# Autodesk Inventor assembly: Male straight header 15p
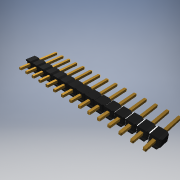
[picture p0: Inventor's stored thumbnail of the model, 180x180]
Saved by Autodesk Inventor 2017 (Build 210142000, 142)
## iProperties
Created: 2017-09-07
Part Number: Male straight header 15p
Document SubType Name: Assembly
Designer: denoqs
Author: denoqs
## Documents named in this file (3)
- E:\Graphic Development\Autodesk Inventor\Inventor output\Arduino things\Arduino header\Male straight header 15p.iam
- E:\Graphic Development\Autodesk Inventor\Inventor output\Arduino things\Arduino header\Housing male header - single.ipt
- E:\Graphic Development\Autodesk Inventor\Inventor output\Arduino things\Arduino header\Pin male header straight - single.ipt
## Components (30 placed, 2 different names)
1. Housing male header - single:1 — Flush:1, Flush:2, Flush:3, Mate:1, Mate:2, Flush:4
2. Pin male header straight - single:1 — Mate:1, Mate:2, Flush:4
3. Housing male header - single:2
4. Pin male header straight - single:2
5. Housing male header - single:3
6. Pin male header straight - single:3
7. Housing male header - single:4
8. Pin male header straight - single:4
9. Housing male header - single:5
10. Pin male header straight - single:5
11. Housing male header - single:6
12. Pin male header straight - single:6
13. Housing male header - single:7
14. Pin male header straight - single:7
15. Housing male header - single:8
16. Pin male header straight - single:8
17. Housing male header - single:9
18. Pin male header straight - single:9
19. Housing male header - single:10
20. Pin male header straight - single:10
21. Housing male header - single:11
22. Pin male header straight - single:11
23. Housing male header - single:12
24. Pin male header straight - single:12
25. Housing male header - single:13
26. Pin male header straight - single:13
27. Housing male header - single:14
28. Pin male header straight - single:14
29. Housing male header - single:15
30. Pin male header straight - single:15
## Component patterns: (15 elements, first: Housing male header - single:1 + Pin male header straight - single:1)
## Relationships (6: Flush 4, Mate 2)
- Flush:1: Housing male header - single:1
- Flush:2: Housing male header - single:1
- Flush:3: Housing male header - single:1
- Mate:1: Housing male header - single:1 ↔ Pin male header straight - single:1
- Mate:2: Housing male header - single:1 ↔ Pin male header straight - single:1
- Flush:4 (-2.54 mm): Housing male header - single:1 ↔ Pin male header straight - single:1
